# Autodesk Inventor assembly: Wall Assembly
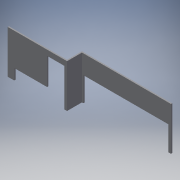
[picture p0: Inventor's stored thumbnail of the model, 180x180]
Saved by Autodesk Inventor 2017 (Build 210142000, 142)
## iProperties
Created: 2017-04-27
Part Number: Wall Assembly
Document SubType Name: Assembly
Designer: hoeflinc
Author: hoeflinc
## Documents named in this file (4)
- P:\me_fsae\Independent Study Battery Pack Deliverables\2016 Inventor Model - Copy\2016 Directory\Electrical\TSI Box\From Chris 2\Wall Assembly.iam
- P:\me_fsae\Independent Study Battery Pack Deliverables\2016 Inventor Model - Copy\2016 Directory\Electrical\TSI Box\From Chris 2\CANIMDWall.ipt
- P:\me_fsae\Independent Study Battery Pack Deliverables\2016 Inventor Model - Copy\2016 Directory\Electrical\TSI Box\From Chris 2\PCBWall.ipt
- P:\me_fsae\Independent Study Battery Pack Deliverables\2016 Inventor Model - Copy\2016 Directory\Electrical\TSI Box\From Chris 2\WallBend.ipt
## Components (3 placed, 3 different names)
1. CANIMDWall:1 — Mate:1, Flush:1, Flush:2
2. PCBWall:1 — Mate:2, Flush:3, Flush:4
3. WallBend:1 — Mate:1, Flush:1, Flush:2, Mate:2, Flush:3, Flush:4
## Relationships (6: Flush 4, Mate 2)
- Mate:1: CANIMDWall:1 ↔ WallBend:1
- Flush:1: CANIMDWall:1 ↔ WallBend:1
- Flush:2: CANIMDWall:1 ↔ WallBend:1
- Mate:2: PCBWall:1 ↔ WallBend:1
- Flush:3: PCBWall:1 ↔ WallBend:1
- Flush:4: PCBWall:1 ↔ WallBend:1
